# Autodesk Inventor assembly: Assembly1
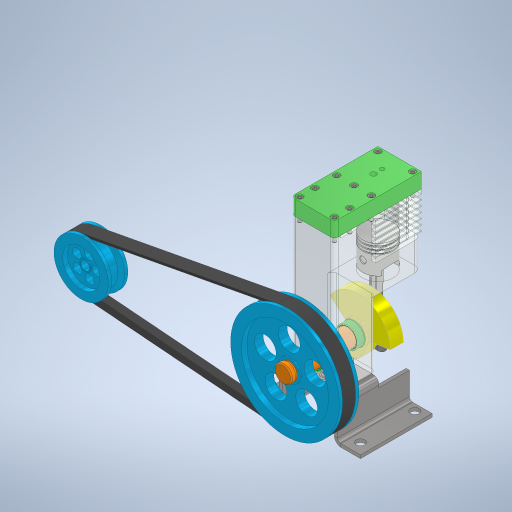
[picture p0: Inventor's stored thumbnail of the model, 512x512]
Saved by Autodesk Inventor 2023 (Build 270158000, 158)
## iProperties
Created: 2023-10-08
Part Number: Assembly1
Document SubType Name: Assembly
Designer: huy20
Author: huy20
## Documents named in this file (17)
- C:\Users\huy20\OneDrive\Máy tính\Inventor\TK Cơ cấu cơ khi\Chi tiết\Máy Nén Khí\Assembly1.iam
- C:\Users\huy20\OneDrive\Máy tính\Inventor\TK Cơ cấu cơ khi\Chi tiết\Máy Nén Khí\Giá đỡ.ipt
- C:\Users\huy20\OneDrive\Máy tính\Inventor\TK Cơ cấu cơ khi\Chi tiết\Máy Nén Khí\Hộp Piston .ipt
- C:\Users\huy20\OneDrive\Máy tính\Inventor\TK Cơ cấu cơ khi\Chi tiết\Máy Nén Khí\Piston.ipt
- C:\Users\huy20\OneDrive\Máy tính\Inventor\TK Cơ cấu cơ khi\Chi tiết\Máy Nén Khí\Piston Pin.ipt
- C:\Users\huy20\OneDrive\Máy tính\Inventor\TK Cơ cấu cơ khi\Chi tiết\Máy Nén Khí\Thanh Truyen 1.ipt
- C:\Users\huy20\OneDrive\Máy tính\Inventor\TK Cơ cấu cơ khi\Chi tiết\Máy Nén Khí\Thanh Truyen.ipt
- C:\Users\huy20\OneDrive\Máy tính\Inventor\TK Cơ cấu cơ khi\Chi tiết\Máy Nén Khí\Crank.ipt
- C:\Users\huy20\OneDrive\Máy tính\Inventor\TK Cơ cấu cơ khi\Chi tiết\Máy Nén Khí\Trục.ipt
- C:\Users\huy20\OneDrive\Máy tính\Inventor\TK Cơ cấu cơ khi\Chi tiết\Máy Nén Khí\Pulley lớn.ipt
- C:\Users\huy20\OneDrive\Máy tính\Inventor\TK Cơ cấu cơ khi\Chi tiết\Máy Nén Khí\Pulley nhỏ.ipt
- C:\Users\huy20\OneDrive\Máy tính\Inventor\TK Cơ cấu cơ khi\Chi tiết\Máy Nén Khí\Nắp hộp piston.ipt
- C:\Users\huy20\OneDrive\Máy tính\Inventor\TK Cơ cấu cơ khi\Chi tiết\Máy Nén Khí\Dây đai.ipt
- C:\Users\huy20\OneDrive\Máy tính\Inventor\TK Cơ cấu cơ khi\Chi tiết\Máy Nén Khí\Vòng Bi.iam
- C:\Users\huy20\OneDrive\Documents\Inventor\Content Center Files\R2023\en-US\CSN 02 1131  B\CSN 02 1131 - M3.5 x 4B.ipt
- C:\Users\huy20\OneDrive\Documents\Inventor\Content Center Files\R2023\en-US\ANSI B18.3.1M(1)\ANSI B18.3.1M - M1.6x0.35 x 8(2).ipt
- C:\Users\huy20\OneDrive\Documents\Inventor\Content Center Files\R2023\en-US\DIN 976-1 B\DIN 976-1 - M2 x 6 - B.ipt
## Components (27 placed, 16 different names)
1. Giá đỡ:1 — Mate:1, Flush:1, Flush:2, Mate:2, Mate:3, Mate:4, Mate:31, Mate:33
2. Hộp Piston :1 — Mate:2, Mate:3, Mate:4, Mate:5, Mate:12, Mate:20, Mate:25, Flush:6, Mate:29, Flush:9, Mate:30, Flush:10, Mate:32, Mate:34
3. Piston:1 — Mate:5, Mate:7, Mate:11, Mate:17
4. Piston Pin:1 — Mate:7, Mate:10, Mate:17
5. Thanh Truyen 1:1 — Mate:8, Mate:9, Flush:3
6. Thanh Truyen:1 — Mate:8, Mate:9, Flush:3, Mate:10, Mate:11, Mate:15, Mate:16, Chuyen Dong, Insert:10, Insert:11
7. Crank:1 — Mate:13, Flush:4, Mate:14, Mate:15, Mate:16, Angle:1
8. Trục:1 — Mate:12, Mate:13, Flush:4, Mate:14, Mate:18, Mate:19, Flush:5, Angle:1, Angle:5
9. Pulley lớn:1 — Mate:18, Mate:19, Flush:5, Chuyen Dong, Mate:26, Flush:7, Flush:8, Angle:3
10. Pulley nhỏ:1 — Mate:26, Mate:28, Angle:3
11. Nắp hộp piston:1 — Mate:20, Mate:25, Flush:6, Mate:35, Mate:36, Mate:37, Mate:38, Mate:39, Mate:40, Mate:41, Mate:42, Mate:43, Mate:44, Mate:45, Mate:46, Mate:47, Mate:48, Mate:49, Mate:50, Mate:51, Mate:52
12. Dây đai:1 — Flush:8, Mate:28
13. Vòng Bi:1 [sub-assembly] — Mate:30, Flush:10, Angle:4
14. Vòng Bi:2 [sub-assembly] — Mate:29, Flush:9, Angle:4, Angle:5
15. CSN 02 1131 B M3.5 x 4:1 — Mate:31, Mate:32
16. CSN 02 1131 B M3.5 x 4:2 — Mate:33, Mate:34
17. DIN 976-1 B M2 x 6:1 — Insert:10
18. DIN 976-1 B M2 x 6:2 — Insert:11
19. Broached Socket Head Cap Screw - Metric M1.6x0.35 x 8:1 — Mate:35, Mate:36
20. Broached Socket Head Cap Screw - Metric M1.6x0.35 x 8:2 — Mate:37, Mate:38
21. Broached Socket Head Cap Screw - Metric M1.6x0.35 x 8:3 — Mate:39, Mate:40
22. Broached Socket Head Cap Screw - Metric M1.6x0.35 x 8:4 — Mate:41, Mate:42
23. Broached Socket Head Cap Screw - Metric M1.6x0.35 x 8:5 — Mate:43, Mate:44
24. Broached Socket Head Cap Screw - Metric M1.6x0.35 x 8:6 — Mate:45, Mate:46
25. Broached Socket Head Cap Screw - Metric M1.6x0.35 x 8:7 — Mate:47, Mate:48
26. Broached Socket Head Cap Screw - Metric M1.6x0.35 x 8:8 — Mate:49, Mate:50
27. Broached Socket Head Cap Screw - Metric M1.6x0.35 x 8:9 — Mate:51, Mate:52
## Relationships (63: Mate 46, Flush 10, Angle 5, Insert 2)
- Mate:1: Giá đỡ:1
- Flush:1: Giá đỡ:1
- Flush:2: Giá đỡ:1
- Mate:2: Giá đỡ:1 ↔ Hộp Piston :1
- Mate:3: Giá đỡ:1 ↔ Hộp Piston :1
- Mate:4: Giá đỡ:1 ↔ Hộp Piston :1
- Mate:5: Hộp Piston :1 ↔ Piston:1
- Mate:7: Piston:1 ↔ Piston Pin:1
- Mate:8: Thanh Truyen 1:1 ↔ Thanh Truyen:1
- Mate:9: Thanh Truyen 1:1 ↔ Thanh Truyen:1
- Flush:3: Thanh Truyen 1:1 ↔ Thanh Truyen:1
- Mate:10: Piston Pin:1 ↔ Thanh Truyen:1
- Mate:11: Piston:1 ↔ Thanh Truyen:1
- Mate:12: Hộp Piston :1 ↔ Trục:1
- Mate:13: Crank:1 ↔ Trục:1
- Flush:4: Crank:1 ↔ Trục:1
- Mate:14: Crank:1 ↔ Trục:1
- Mate:15: Thanh Truyen:1 ↔ Crank:1
- Mate:16: Thanh Truyen:1 ↔ Crank:1
- Mate:17: Piston:1 ↔ Piston Pin:1
- Mate:18: Trục:1 ↔ Pulley lớn:1
- Mate:19: Trục:1 ↔ Pulley lớn:1
- Flush:5: Trục:1 ↔ Pulley lớn:1
- Angle:1 (0 deg): Crank:1 ↔ Trục:1
- Chuyen Dong [Angle] (3252 deg): Thanh Truyen:1 ↔ Pulley lớn:1
- Mate:20: Hộp Piston :1 ↔ Nắp hộp piston:1
- Mate:25: Hộp Piston :1 ↔ Nắp hộp piston:1
- Flush:6: Hộp Piston :1 ↔ Nắp hộp piston:1
- Mate:26: Pulley lớn:1 ↔ Pulley nhỏ:1
- Flush:7: Pulley lớn:1
- Flush:8: Pulley lớn:1 ↔ Dây đai:1
- Mate:28: Pulley nhỏ:1 ↔ Dây đai:1
- Angle:3 (0 deg): Pulley lớn:1 ↔ Pulley nhỏ:1
- Mate:29: Hộp Piston :1 ↔ Vòng Bi:2
- Flush:9: Hộp Piston :1 ↔ Vòng Bi:2
- Mate:30: Hộp Piston :1 ↔ Vòng Bi:1
- Flush:10: Hộp Piston :1 ↔ Vòng Bi:1
- Angle:4 (0 deg): Vòng Bi:1 ↔ Vòng Bi:2
- Angle:5 (0 deg): Trục:1 ↔ Vòng Bi:2
- Mate:31: Giá đỡ:1 ↔ CSN 02 1131 B M3.5 x 4:1
- Mate:32: Hộp Piston :1 ↔ CSN 02 1131 B M3.5 x 4:1
- Mate:33: Giá đỡ:1 ↔ CSN 02 1131 B M3.5 x 4:2
- Mate:34: Hộp Piston :1 ↔ CSN 02 1131 B M3.5 x 4:2
- Insert:10 (-5.7546 mm): Thanh Truyen:1 ↔ DIN 976-1 B M2 x 6:1
- Insert:11 (-5.7546 mm): Thanh Truyen:1 ↔ DIN 976-1 B M2 x 6:2
- Mate:35: Nắp hộp piston:1 ↔ Broached Socket Head Cap Screw - Metric M1.6x0.35 x 8:1
- Mate:36: Nắp hộp piston:1 ↔ Broached Socket Head Cap Screw - Metric M1.6x0.35 x 8:1
- Mate:37: Nắp hộp piston:1 ↔ Broached Socket Head Cap Screw - Metric M1.6x0.35 x 8:2
- Mate:38: Nắp hộp piston:1 ↔ Broached Socket Head Cap Screw - Metric M1.6x0.35 x 8:2
- Mate:39: Nắp hộp piston:1 ↔ Broached Socket Head Cap Screw - Metric M1.6x0.35 x 8:3
- Mate:40: Nắp hộp piston:1 ↔ Broached Socket Head Cap Screw - Metric M1.6x0.35 x 8:3
- Mate:41: Nắp hộp piston:1 ↔ Broached Socket Head Cap Screw - Metric M1.6x0.35 x 8:4
- Mate:42: Nắp hộp piston:1 ↔ Broached Socket Head Cap Screw - Metric M1.6x0.35 x 8:4
- Mate:43: Nắp hộp piston:1 ↔ Broached Socket Head Cap Screw - Metric M1.6x0.35 x 8:5
- Mate:44: Nắp hộp piston:1 ↔ Broached Socket Head Cap Screw - Metric M1.6x0.35 x 8:5
- Mate:45: Nắp hộp piston:1 ↔ Broached Socket Head Cap Screw - Metric M1.6x0.35 x 8:6
- Mate:46: Nắp hộp piston:1 ↔ Broached Socket Head Cap Screw - Metric M1.6x0.35 x 8:6
- Mate:47: Nắp hộp piston:1 ↔ Broached Socket Head Cap Screw - Metric M1.6x0.35 x 8:7
- Mate:48: Nắp hộp piston:1 ↔ Broached Socket Head Cap Screw - Metric M1.6x0.35 x 8:7
- Mate:49: Nắp hộp piston:1 ↔ Broached Socket Head Cap Screw - Metric M1.6x0.35 x 8:8
- Mate:50: Nắp hộp piston:1 ↔ Broached Socket Head Cap Screw - Metric M1.6x0.35 x 8:8
- Mate:51: Nắp hộp piston:1 ↔ Broached Socket Head Cap Screw - Metric M1.6x0.35 x 8:9
- Mate:52: Nắp hộp piston:1 ↔ Broached Socket Head Cap Screw - Metric M1.6x0.35 x 8:9
